# Autodesk Inventor assembly: PlanetaryGearmotor
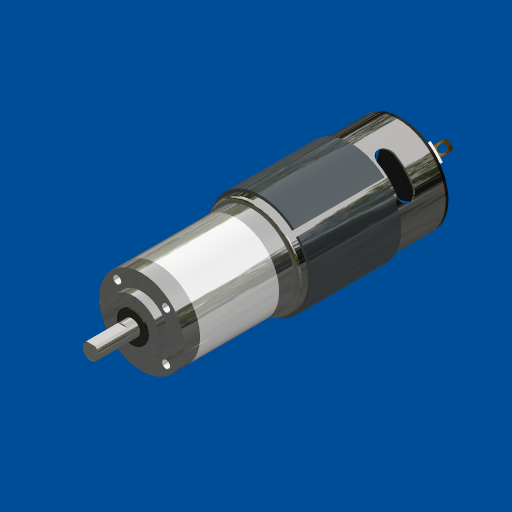
[picture p0: Inventor's stored thumbnail of the model, 512x512]
Saved by Autodesk Inventor 2023 (Build 270158030, 158C)
## iProperties
Created: 2023-02-26
Part Number: PlanetaryGearmotor
Document SubType Name: Assembly
Designer: kumpu
Mass: 380 g
Surface Area: 225.636 cm^2
Volume: 42.1455 cm^3
Author: kumpu
## Documents named in this file (3)
- C:\Users\kumpu\Documents\SBU\CAD\SBRT\Robocup Rescue\Arm\final\PlanetaryGearmotor.iam
- C:\Users\kumpu\Documents\SBU\CAD\SBRT\Robocup Rescue\Arm\final\550Motor.ipt
- C:\Users\kumpu\Documents\SBU\CAD\SBRT\Robocup Rescue\Arm\final\PlanetaryGearbox.ipt
## Components (2 placed, 2 different names)
1. 550Motor:1 — Angle:1, Insert:1
2. PlanetaryGearbox:1 — Flush:2, Flush:1, Flush:3, Insert:1
## Relationships (5: Flush 3, Angle 1, Insert 1)
- Flush:2: PlanetaryGearbox:1
- Flush:1: PlanetaryGearbox:1
- Flush:3: PlanetaryGearbox:1
- Angle:1 (45 deg): 550Motor:1
- Insert:1: 550Motor:1 ↔ PlanetaryGearbox:1
